# Autodesk Inventor assembly: Мостики
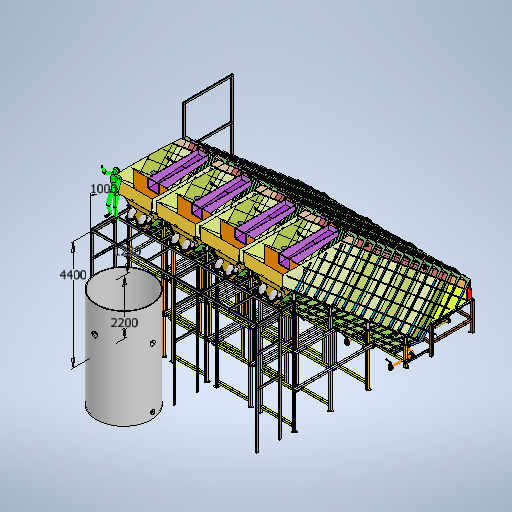
[picture p0: Inventor's stored thumbnail of the model, 512x512]
Saved by Autodesk Inventor 2025 (Build 290162010, 162A)
## iProperties
Created: 2025-01-27
Part Number: Мостики
Document SubType Name: Assembly
Designer: admin
Author: admin
## Documents named in this file (7)
- C:\Users\admin\YandexDisk-badmisterfox\домашниий пк\Inventor\Manturovo\Manturovo_Se-clar\Мостики.iam
- C:\Users\admin\YandexDisk-badmisterfox\домашниий пк\Inventor\Manturovo\Manturovo_Se-clar\ASY MSC 002 отстойник осветлитель.iam
- C:\Users\admin\YandexDisk-badmisterfox\домашниий пк\Inventor\Manturovo\Manturovo_Se-clar\human 01\ч ASY human dummy 01.iam
- C:\Users\admin\YandexDisk-badmisterfox\домашниий пк\Inventor\Manturovo\Manturovo_Se-clar\ASY MSC Платформа отстойников.iam
- C:\Users\admin\YandexDisk-badmisterfox\домашниий пк\Inventor\Manturovo\Manturovo_Se-clar\ASY MSC Опора №1 платф. отст..iam
- C:\Users\admin\YandexDisk-badmisterfox\домашниий пк\Inventor\Manturovo\Manturovo_Se-clar\ASY MSC Опора №2 платф. отст..iam
- C:\Users\admin\YandexDisk-badmisterfox\домашниий пк\Inventor\Manturovo\Manturovo_Se-clar\Габаритные емкости для Димы\Отстойник промывных вод.ipt
## Components (11 placed, 6 different names)
1. ASY MSC 002 отстойник осветлитель:1 [sub-assembly] — Flush:1, Flush:2, Flush:3, Flush:4, Rigid:1, Flush:5, Mate:1, Mate:2
2. ASY MSC 002 отстойник осветлитель:2 [sub-assembly] — Rigid:1, Rigid:2, Mate:4, Flush:6
3. ASY MSC 002 отстойник осветлитель:3 [sub-assembly] — Rigid:3
4. ASY MSC 002 отстойник осветлитель:4 [sub-assembly] — Rigid:2, Rigid:3
5. ч ASY human dummy 01:1 [sub-assembly] — Flush:1
6. ASY MSC Платформа отстойников:1 [sub-assembly] — Flush:5, Mate:1, Mate:2, Rigid:4, Rigid:5, Rigid:6
7. ASY MSC Опора №1 платф. отст.:1 [sub-assembly] — Rigid:4
8. ASY MSC Опора №1 платф. отст.:2 [sub-assembly] — Rigid:5
9. ASY MSC Опора №2 платф. отст.:1 [sub-assembly]
10. ASY MSC Опора №1 платф. отст.:3 [sub-assembly] — Rigid:6
11. Отстойник промывных вод:1 — Mate:3, Mate:4, Flush:6
## Relationships (16: Flush 6, WeldJoint 6, Mate 4)
- Flush:1 (4500 mm): ASY MSC 002 отстойник осветлитель:1 ↔ ч ASY human dummy 01:1
- Flush:2: ASY MSC 002 отстойник осветлитель:1
- Flush:3: ASY MSC 002 отстойник осветлитель:1
- Flush:4: ASY MSC 002 отстойник осветлитель:1
- Rigid:1 [WeldJoint] (50 mm): ASY MSC 002 отстойник осветлитель:1 ↔ ASY MSC 002 отстойник осветлитель:2
- Rigid:2 [WeldJoint] (50 mm): ASY MSC 002 отстойник осветлитель:2 ↔ ASY MSC 002 отстойник осветлитель:4
- Rigid:3 [WeldJoint] (50 mm): ASY MSC 002 отстойник осветлитель:3 ↔ ASY MSC 002 отстойник осветлитель:4
- Flush:5 (20 mm): ASY MSC 002 отстойник осветлитель:1 ↔ ASY MSC Платформа отстойников:1
- Mate:1 (50 mm): ASY MSC 002 отстойник осветлитель:1 ↔ ASY MSC Платформа отстойников:1
- Mate:2: ASY MSC 002 отстойник осветлитель:1 ↔ ASY MSC Платформа отстойников:1
- Rigid:4 [WeldJoint]: ASY MSC Платформа отстойников:1 ↔ ASY MSC Опора №1 платф. отст.:1
- Rigid:5 [WeldJoint]: ASY MSC Платформа отстойников:1 ↔ ASY MSC Опора №1 платф. отст.:2
- Rigid:6 [WeldJoint]: ASY MSC Платформа отстойников:1 ↔ ASY MSC Опора №1 платф. отст.:3
- Mate:3: Отстойник промывных вод:1
- Mate:4 (1900 mm): ASY MSC 002 отстойник осветлитель:2 ↔ Отстойник промывных вод:1
- Flush:6 (200 mm): ASY MSC 002 отстойник осветлитель:2 ↔ Отстойник промывных вод:1
